# Autodesk Inventor assembly: ChestFrameDesign
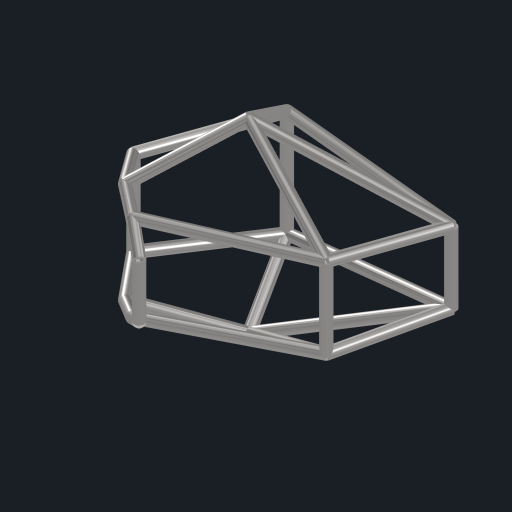
[picture p0: Inventor's stored thumbnail of the model, 512x512]
Saved by Autodesk Inventor 2023 (Build 270158000, 158)
## iProperties
Created: 2023-12-08
Part Number: ChestFrameDesign
Document SubType Name: Assembly
Designer: valer
_SolveAssemblyDoc: Frame Generator Solve Assembly
_Version: 15.0.0
Author: valer
## Documents named in this file (3)
- C:\Users\valer\Desktop\str1ker\design\ChestFrameDesign.iam
- C:\Users\valer\Desktop\str1ker\design\ChestFrameDesign.ipt
- C:\Users\valer\Desktop\str1ker\cad\Chest\Frame.iam
## Components (2 placed, 2 different names)
1. ChestFrameDesign:1 — Mate:1
2. Frame:1 [sub-assembly]
## Relationships (1: Mate 1)
- Mate:1: ChestFrameDesign:1
